# Autodesk Inventor assembly: IndexerA
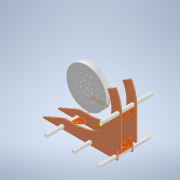
[picture p0: Inventor's stored thumbnail of the model, 180x180]
Saved by Autodesk Inventor 2020 (Build 240168000, 168)
## iProperties
Created: 2020-01-19
Part Number: IndexerA
Document SubType Name: Assembly
Designer: srini
Author: srini
## Documents named in this file (7)
- C:\Users\srini\Documents\FRC\2020\IntakeShooter\IndexerA.iam
- C:\Users\srini\Documents\FRC\2020\IntakeShooter\CenterIndexerWheel.ipt
- C:\Users\srini\Documents\FRC\2020\IntakeShooter\OuterWheelIndexer.ipt
- C:\Users\srini\Documents\FRC\2020\IntakeShooter\OuterWheelIndexer_MIR.ipt
- C:\Users\srini\Documents\FRC\2020\IntakeShooter\1x1x20.25.ipt
- C:\Users\srini\Documents\FRC\2020\IntakeShooter\IndexerSpacer5_5.ipt
- C:\Users\srini\Documents\FRC\2020\IntakeShooter\IndexerSpacer5_5_2.ipt
## Components (12 placed, 6 different names)
1. CenterIndexerWheel:1 — Mate:1, Mate:4, Flush:3
2. OuterWheelIndexer:1 — Mate:1, Flush:4, Mate:5, Mate:6, Mate:7, Mate:11, Mate:12, Mate:13, Mate:14, Mate:15, Mate:16, Mate:17, Mate:20
3. OuterWheelIndexer_MIR:1 — Mate:4, Mate:8, Mate:10, Mate:19
4. 1x1x20.25:1 — Insert:1, Insert:2, Mate:6, Mate:7, Insert:5, Insert:6
5. 1x1x20.25:2 — Insert:3, Insert:4, Mate:8, Mate:14, Mate:19, Mate:20
6. 1x1x20.25:3 — Insert:7, Insert:8, Mate:11, Mate:12
7. IndexerSpacer5_5:1 — Insert:1, Insert:2, Mate:5
8. IndexerSpacer5_5:2 — Insert:3, Insert:4, Mate:10
9. IndexerSpacer5_5:3 — Insert:7, Insert:8, Mate:13
10. IndexerSpacer5_5:4 — Insert:5, Insert:6
11. 1x1x20.25:4 — Mate:15, Mate:16, Insert:9, Insert:10
12. IndexerSpacer5_5_2:1 — Insert:9, Insert:10, Mate:17
## Relationships (28: Mate 16, Insert 10, Flush 2)
- Mate:1 (44.45 mm): CenterIndexerWheel:1 ↔ OuterWheelIndexer:1
- Mate:4 (44.45 mm): CenterIndexerWheel:1 ↔ OuterWheelIndexer_MIR:1
- Flush:3: CenterIndexerWheel:1
- Flush:4: OuterWheelIndexer:1
- Insert:1: 1x1x20.25:1 ↔ IndexerSpacer5_5:1
- Insert:2: 1x1x20.25:1 ↔ IndexerSpacer5_5:1
- Mate:5: OuterWheelIndexer:1 ↔ IndexerSpacer5_5:1
- Mate:6: OuterWheelIndexer:1 ↔ 1x1x20.25:1
- Mate:7: OuterWheelIndexer:1 ↔ 1x1x20.25:1
- Insert:3: 1x1x20.25:2 ↔ IndexerSpacer5_5:2
- Insert:4: 1x1x20.25:2 ↔ IndexerSpacer5_5:2
- Insert:5: 1x1x20.25:1 ↔ IndexerSpacer5_5:4
- Insert:6: 1x1x20.25:1 ↔ IndexerSpacer5_5:4
- Mate:8: OuterWheelIndexer_MIR:1 ↔ 1x1x20.25:2
- Mate:10: OuterWheelIndexer_MIR:1 ↔ IndexerSpacer5_5:2
- Insert:7: 1x1x20.25:3 ↔ IndexerSpacer5_5:3
- Insert:8: 1x1x20.25:3 ↔ IndexerSpacer5_5:3
- Mate:11: OuterWheelIndexer:1 ↔ 1x1x20.25:3
- Mate:12: OuterWheelIndexer:1 ↔ 1x1x20.25:3
- Mate:13: OuterWheelIndexer:1 ↔ IndexerSpacer5_5:3
- Mate:14: OuterWheelIndexer:1 ↔ 1x1x20.25:2
- Mate:15: OuterWheelIndexer:1 ↔ 1x1x20.25:4
- Mate:16: OuterWheelIndexer:1 ↔ 1x1x20.25:4
- Insert:9: 1x1x20.25:4 ↔ IndexerSpacer5_5_2:1
- Insert:10: 1x1x20.25:4 ↔ IndexerSpacer5_5_2:1
- Mate:17: OuterWheelIndexer:1 ↔ IndexerSpacer5_5_2:1
- Mate:19: OuterWheelIndexer_MIR:1 ↔ 1x1x20.25:2
- Mate:20: OuterWheelIndexer:1 ↔ 1x1x20.25:2
